# Autodesk Inventor assembly: 775pro_1_E_1-2inHex
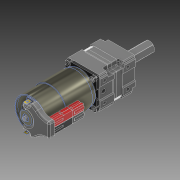
[picture p0: Inventor's stored thumbnail of the model, 180x180]
Saved by Autodesk Inventor 2022 (Build 260153000, 153)
## iProperties
Created: 2018-08-19
Part Number: 775pro_1_E_1-2inHex
Document SubType Name: Assembly
Mass: 1123.04 g
Surface Area: 1203.25 cm^2
Volume: 285.054 cm^3
Density: 3.93975 g/cm^3
## Documents named in this file (10)
- C:\Users\Cal\Desktop\Robotics\Design\Collaborative\Collaborative Parts Library\General Gearboxes\Planetaries\Versaplanetary\VersaPlanetary\775pro, 1 Stages, Encoder, 1-2in Hex Output.iam
- C:\Users\Cal\Desktop\Robotics\Design\Collaborative\Collaborative Parts Library\General Gearboxes\Planetaries\Versaplanetary\Intermediate Stages\VP Encoder.iam
- C:\Users\Cal\Desktop\Robotics\Design\Collaborative\Collaborative Parts Library\General Gearboxes\Planetaries\Versaplanetary\V2 Stages\V2 Input Stage.iam
- C:\Users\Cal\Desktop\Robotics\Design\Collaborative\Collaborative Parts Library\General Gearboxes\Planetaries\Versaplanetary\Screws\8-32 x 1.75in Screw.ipt
- C:\Users\Cal\Desktop\Robotics\Design\Collaborative\Collaborative Parts Library\Power Transfer\Bearings and Bushings\Bearings\6902ZZ.ipt
- E:\Middleton Robotics\Collaborative Robots\Colaborative Part Library\General Gearboxes\Planetaries\Versaplanetary\V2 Stages\V2 Output Stage.iam
- E:\Middleton Robotics\Collaborative Robots\Collaborative Part Library\Power Transfer\Bearings.ipt
- C:\Users\Cal\Desktop\Robotics\Design\Collaborative\Collaborative Parts Library\General Gearboxes\Planetaries\Versaplanetary\V2 Stages\V2 Output Stage\VP V2 Output Stage 1-2in Hex.iam
- C:\Users\Cal\Desktop\Robotics\Design\Collaborative\Collaborative Parts Library\General Gearboxes\Planetaries\Versaplanetary\V2 Stages\V2 Input Stage\VP 775pro Input.iam
- C:\Users\Cal\Desktop\Robotics\Design\Collaborative\Collaborative Parts Library\General Gearboxes\Planetaries\Versaplanetary\VersaPlanetary.iam
## Components (7 placed, 5 different names)
1. VP V2 Output Stage 1-2in Hex:1 [sub-assembly] — EncoderConstraint1, EncoderConstraint2, EncoderConstraint3, EncoderBasicInputMate2, Insert:25
2. VP Encoder:1 [sub-assembly] — EncoderConstraint1, EncoderConstraint2, EncoderConstraint3, EncoderBasicInputMate1
3. VP 775pro Input:1 [sub-assembly] — EncoderBasicInputMate1, EncoderBasicInputMate2, Insert:8, Insert:9
4. 8-32 x 1.75in Screw:1 — Insert:8
5. 8-32 x 1.75in Screw:2 — Insert:9
6. 6902ZZ:1
7. 6902ZZ:2 — Insert:25
## Relationships (8: Insert 4, Mate 2, Angle 1, Flush 1)
- EncoderConstraint1 [Mate]: VP V2 Output Stage 1-2in Hex:1 ↔ VP Encoder:1
- EncoderConstraint2 [Mate]: VP V2 Output Stage 1-2in Hex:1 ↔ VP Encoder:1
- EncoderConstraint3 [Angle] (0 deg): VP V2 Output Stage 1-2in Hex:1 ↔ VP Encoder:1
- EncoderBasicInputMate1 [Insert]: VP Encoder:1 ↔ VP 775pro Input:1
- EncoderBasicInputMate2 [Flush]: VP V2 Output Stage 1-2in Hex:1 ↔ VP 775pro Input:1
- Insert:8: VP 775pro Input:1 ↔ 8-32 x 1.75in Screw:1
- Insert:9: VP 775pro Input:1 ↔ 8-32 x 1.75in Screw:2
- Insert:25: VP V2 Output Stage 1-2in Hex:1 ↔ 6902ZZ:2
